# Autodesk Inventor assembly: złożenie_840
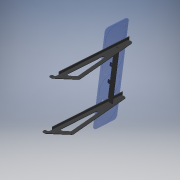
[picture p0: Inventor's stored thumbnail of the model, 180x180]
Saved by Autodesk Inventor 2017 (Build 210142000, 142)
## iProperties
Part Number: złożenie_840
Material: Ogólny
Document SubType Name: Assembly
Designer: patry
Author: patry
## Documents named in this file (5)
- C:\Users\patry\Desktop\Mocowanie_wykrywacz\złożenie_840.iam
- C:\Users\patry\Desktop\Mocowanie_wykrywacz\nowy_bok.ipt
- C:\Users\patry\Desktop\Mocowanie_wykrywacz\poprz_teownik.ipt
- C:\Users\patry\Desktop\Mocowanie_wykrywacz\poprz_690.ipt
- C:\Users\patry\Desktop\Mocowanie_wykrywacz\Cewki_840.ipt
## Components (6 placed, 4 different names)
1. nowy_bok:1 — Zestawiający:1, Zestawiający:2, Zestawiający:3, Zestawiający:7, Zestawiający:13
2. poprz_teownik:1 — Zestawiający:1, Zestawiający:2, Zestawiający:3, Równoległy:1, Równoległy:2
3. nowy_bok:2 — Zestawiający:7, Zestawiający:8, Zestawiający:10
4. poprz_teownik:2 — Równoległy:1, Równoległy:2, Zestawiający:9
5. poprz_690:1 — Zestawiający:8, Zestawiający:9, Zestawiający:10, Zestawiający:11, Zestawiający:12
6. Cewki_840:1 — Zestawiający:11, Zestawiający:12, Zestawiający:13
## Relationships (15: Mate 13, Flush 2)
- Zestawiający:1 [Mate]: nowy_bok:1 ↔ poprz_teownik:1
- Zestawiający:2 [Mate]: nowy_bok:1 ↔ poprz_teownik:1
- Zestawiający:3 [Mate] (0.5 mm): nowy_bok:1 ↔ poprz_teownik:1
- [Mate]: nowy_bok:2 ↔ poprz_teownik:2
- [Mate]: nowy_bok:2 ↔ poprz_teownik:2
- [Mate] (0.5 mm): nowy_bok:2 ↔ poprz_teownik:2
- Zestawiający:7 [Mate] (450 mm): nowy_bok:1 ↔ nowy_bok:2
- Równoległy:1 [Flush]: poprz_teownik:1 ↔ poprz_teownik:2
- Równoległy:2 [Flush]: poprz_teownik:1 ↔ poprz_teownik:2
- Zestawiający:8 [Mate]: nowy_bok:2 ↔ poprz_690:1
- Zestawiający:9 [Mate]: poprz_teownik:2 ↔ poprz_690:1
- Zestawiający:10 [Mate] (0.5 mm): nowy_bok:2 ↔ poprz_690:1
- Zestawiający:11 [Mate]: poprz_690:1 ↔ Cewki_840:1
- Zestawiający:12 [Mate]: poprz_690:1 ↔ Cewki_840:1
- Zestawiający:13 [Mate]: nowy_bok:1 ↔ Cewki_840:1
## Named parameters: d3_d2 = 0.5 mm, d4_d0 = 0 mm, d5_d1 = 0 mm
